# Autodesk Inventor assembly: Spinn5_Enclosure
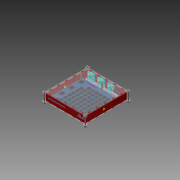
[picture p0: Inventor's stored thumbnail of the model, 180x180]
Saved by Autodesk Inventor 2015 SP1 (Build 190203100, 203)
## iProperties
Created: 2014-08-07
Part Number: Spinn5_Enclosure
Document SubType Name: Assembly
Designer: Patrick Camilleri
Author: Patrick Camilleri
## Documents named in this file (11)
- C:\Users\Patrick\CAD\Spin5 Enclosure\Spinn5_Enclosure.iam
- C:\Users\Patrick\CAD\Spin5 Enclosure\BasePlate.ipt
- C:\Users\Patrick\CAD\Spin5 Enclosure\SidePanel.ipt
- C:\Users\Patrick\CAD\Spin5 Enclosure\SidePanelFans2.iam
- C:\Users\Patrick\CAD\Spin5 Enclosure\BoltAssembly.iam
- C:\Users\Patrick\CAD\Spin5 Enclosure\Stopper.ipt
- C:\Users\Patrick\CAD\Spin5 PowerPcb\Imported Components\Spinn5Power\Spinn5Power.iam
- C:\Users\Patrick\CAD\Spin5 Board\Spin5 Inventor Simple 2\Imported Components\spin5v1_simple_2\spin5v1_simple_2.iam
- C:\Users\Patrick\CAD\Spin5 Enclosure\SidePanel_v2_left.iam
- C:\Users\Patrick\CAD\Spin5 Enclosure\SidePanel_v2_right.iam
- C:\Users\Patrick\CAD\Spin5 Enclosure\TopPlate2.ipt
## Components (13 placed, 10 different names)
1. BasePlate:1 — Rigid:19, Rigid:29, Rigid:32, Rigid:33, Rigid:34
2. SidePanel:1 — Rigid:32
3. BoltAssembly:1 [sub-assembly]
4. BoltAssembly:2 [sub-assembly]
5. BoltAssembly:3 [sub-assembly]
6. BoltAssembly:4 [sub-assembly]
7. Stopper:1 — Rigid:19
8. spin5v1_simple_2:1 [sub-assembly] — Mate:5, Mate:6, Mate:7
9. SidePanelFans2:1 [sub-assembly] — Rigid:34
10. Spinn5Power:1 [sub-assembly] — Mate:5, Mate:6, Mate:7
11. SidePanel_v2_left:1 [sub-assembly] — Rigid:29
12. SidePanel_v2_right:1 [sub-assembly] — Rigid:33
13. TopPlate2:1
## Relationships (8: WeldJoint 5, Mate 3)
- Rigid:19 [WeldJoint]: BasePlate:1 ↔ Stopper:1
- Rigid:29 [WeldJoint]: BasePlate:1 ↔ SidePanel_v2_left:1
- Mate:5: spin5v1_simple_2:1 ↔ Spinn5Power:1
- Mate:6: spin5v1_simple_2:1 ↔ Spinn5Power:1
- Mate:7: spin5v1_simple_2:1 ↔ Spinn5Power:1
- Rigid:32 [WeldJoint]: BasePlate:1 ↔ SidePanel:1
- Rigid:33 [WeldJoint]: BasePlate:1 ↔ SidePanel_v2_right:1
- Rigid:34 [WeldJoint]: BasePlate:1 ↔ SidePanelFans2:1
